# Autodesk Inventor assembly: 00090C
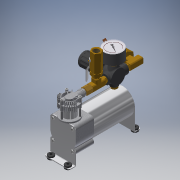
[picture p0: Inventor's stored thumbnail of the model, 180x180]
Saved by Autodesk Inventor 2016 (Build 200138000, 138)
## iProperties
Category: Pneumatics
Company: Autodesk Inc.
Created: 2015-12-06
Part Number: 00090C
Document SubType Name: Assembly
Designer: Autodesk Inc.
Catalog Web Link: http://www.viaircorp.com/OffRoad/90C.html
Description: Air Compressor 90C
Vendor: VIAIR
Author: Autodesk Inc.
## Documents named in this file (18)
- E:\Improved  2011 Robot\FRC KOP 2016\Pneumatics\Pneu_Compressor_0090C.iam
- E:\Improved  2011 Robot\FRC KOP 2016\Pneumatics\Parts\Pneumatics_VIAIR_0090_01.ipt
- E:\Improved  2011 Robot\FRC KOP 2016\Pneumatics\Parts\Pneumatics_VIAIR_0090_02.ipt
- E:\Improved  2011 Robot\FRC KOP 2016\Pneumatics\Parts\Pneumatics_VIAIR_00090_03.ipt
- E:\Improved  2011 Robot\FRC KOP 2016\Pneumatics\Parts\Pneumatics_VIAIR_0090_04.ipt
- E:\Improved  2011 Robot\FRC KOP 2016\Pneumatics\Parts\Union_62C-2.ipt
- E:\Improved  2011 Robot\FRC KOP 2016\Pneumatics\Parts\Pneumatic_VIAIR_Fitting.ipt
- E:\Improved  2011 Robot\FRC KOP 2016\Pneumatics\Parts\Pneumatics_VIAIR_00090_02.ipt
- E:\Improved  2011 Robot\FRC KOP 2016\Miscellaneous\Parts\ANSI B18.3 - 5-40 UNC - 1.5(31).ipt
- E:\Improved  2011 Robot\FRC KOP 2016\Miscellaneous\Parts\ANSI B18.3 - 6-32 UNC - UNC - 0.25(1).ipt
- E:\Improved  2011 Robot\FRC KOP 2016\Miscellaneous\Parts\ANSI B18.6.3 - 8-32 UNC - 1.25(30).ipt
- E:\Improved  2011 Robot\FRC KOP 2016\Pneumatics\Parts\Pneumatic_VIAIAR_00090_05.ipt
- E:\Improved  2011 Robot\FRC KOP 2016\Pneumatics\Pneu_Norgren_R07-100-RNEA.iam
- E:\Improved  2011 Robot\FRC KOP 2016\Pneumatics\Pneu_Plug_218P-2.ipt
- E:\Improved  2011 Robot\FRC KOP 2016\Pneumatics\Pneu_Parker_MV709-2.ipt
- E:\Improved  2011 Robot\FRC KOP 2016\Pneumatics\Pneu_Switch_SM-2B-115R.ipt
- E:\Improved  2011 Robot\FRC KOP 2016\Pneumatics\fc16-104_7.ipt
- E:\Improved  2011 Robot\FRC KOP 2016\Pneumatics\Pneu_Nipple_216P-2.ipt
## Components (29 placed, 17 different names)
1. Pneumatics_VIAIR_0090_01:1 — Mate:1, Flush:1, Flush:2, Mate:4, Angle:1, Mate:14, Mate:15, Mate:16, Mate:17, Mate:18, Mate:19, Mate:20, Mate:21, Angle:3, Mate:23, Mate:24, Flush:9, Flush:10, Mate:30, Mate:31
2. Pneumatics_VIAIR_0090_02:1 — Mate:1, Flush:1, Flush:2, Flush:3, Mate:2, Mate:3, Angle:2, Mate:29
3. Pneumatics_VIAIR_00090_03:1 — Flush:3, Mate:27, Mate:28, Mate:29
4. Pneumatics_VIAIR_0090_04:1 — Mate:2, Mate:3, Angle:2, Mate:6, Mate:7, Mate:8, Mate:9, Mate:10, Mate:11, Mate:12, Mate:13
5. Union_62C-2:1
6. Pneumatic_VIAIR_Fitting:1 — Mate:6, Mate:7, Mate:38, Mate:39
7. Pneumatics_VIAIR_00090_02:1 — Insert:1, Insert:2, Mate:25, Mate:26, Mate:27, Mate:28, Flush:9, Flush:10, Angle:4, Mate:32, Mate:33
8. Hexagon Socket Head Cap Screw - Inch No. 5 - 40 UNC - 1 1/2:1 — Mate:8, Mate:9
9. Hexagon Socket Head Cap Screw - Inch No. 5 - 40 UNC - 1 1/2:2 — Mate:10, Mate:11
10. Hexagon Socket Head Cap Screw - Inch No. 5 - 40 UNC - 1 1/2:3 — Mate:12, Mate:13
11. Hexagon Socket Button Head Cap Screw - Inch 6 - 32 x 1/4:1 — Mate:14, Mate:15
12. Hexagon Socket Button Head Cap Screw - Inch 6 - 32 x 1/4:2 — Mate:16, Mate:17
13. Hexagon Socket Button Head Cap Screw - Inch 6 - 32 x 1/4:3 — Mate:18, Mate:19
14. Hexagon Socket Button Head Cap Screw - Inch 6 - 32 x 1/4:4 — Mate:20, Mate:21
15. Indented Large Hex Head Machine Screw - Inch 8-32 UNC - 1.25:1 — Insert:1
16. Indented Large Hex Head Machine Screw - Inch 8-32 UNC - 1.25:2 — Insert:2
17. Pneumatic_VIAIAR_00090_05:1 — Mate:23, Mate:24
18. Pneumatic_VIAIAR_00090_05:2 — Mate:25, Mate:26, Angle:4
19. Pneumatic_VIAIAR_00090_05:3 — Mate:30, Mate:31
20. Pneumatic_VIAIAR_00090_05:4 — Mate:32, Mate:33
21. Pneu_Norgren_R07-100-RNEA:1 [sub-assembly] — Mate:36, Mate:37, Mate:43, Mate:44, Mate:49, Mate:50
22. Pneu_Plug_218P-2:1 — Mate:36, Mate:37
23. Pneu_Parker_MV709-2:1 — Mate:47, Mate:48
24. Pneu_Switch_SM-2B-115R:1 — Mate:53, Mate:54
25. fc16-104_7:1 — Mate:38, Mate:39, Mate:40, Mate:41, Mate:42, Mate:45, Mate:46
26. fc16-104_7:2 — Mate:51, Mate:52, Mate:53, Mate:54
27. Pneu_Nipple_216P-2:1 — Mate:40, Mate:41, Mate:42, Mate:43, Mate:44
28. Pneu_Nipple_216P-2:2 — Mate:45, Mate:46, Mate:47, Mate:48
29. Pneu_Nipple_216P-2:3 — Mate:49, Mate:50, Mate:51, Mate:52
## Relationships (64: Mate 52, Flush 6, Angle 4, Insert 2)
- Mate:1: Pneumatics_VIAIR_0090_01:1 ↔ Pneumatics_VIAIR_0090_02:1
- Flush:1: Pneumatics_VIAIR_0090_01:1 ↔ Pneumatics_VIAIR_0090_02:1
- Flush:2: Pneumatics_VIAIR_0090_01:1 ↔ Pneumatics_VIAIR_0090_02:1
- Flush:3: Pneumatics_VIAIR_0090_02:1 ↔ Pneumatics_VIAIR_00090_03:1
- Mate:2: Pneumatics_VIAIR_0090_02:1 ↔ Pneumatics_VIAIR_0090_04:1
- Mate:3: Pneumatics_VIAIR_0090_02:1 ↔ Pneumatics_VIAIR_0090_04:1
- Mate:4: Pneumatics_VIAIR_0090_01:1
- Mate:5
- Angle:1 (90 deg): Pneumatics_VIAIR_0090_01:1
- Flush:5 (-69.977 mm)
- Angle:2 (0 deg): Pneumatics_VIAIR_0090_02:1 ↔ Pneumatics_VIAIR_0090_04:1
- Mate:6: Pneumatics_VIAIR_0090_04:1 ↔ Pneumatic_VIAIR_Fitting:1
- Mate:7 (1.27 mm): Pneumatics_VIAIR_0090_04:1 ↔ Pneumatic_VIAIR_Fitting:1
- Mate:9: Pneumatics_VIAIR_0090_04:1 ↔ Hexagon Socket Head Cap Screw - Inch No. 5 - 40 UNC - 1 1/2:1
- Mate:11: Pneumatics_VIAIR_0090_04:1 ↔ Hexagon Socket Head Cap Screw - Inch No. 5 - 40 UNC - 1 1/2:2
- Mate:13: Pneumatics_VIAIR_0090_04:1 ↔ Hexagon Socket Head Cap Screw - Inch No. 5 - 40 UNC - 1 1/2:3
- Mate:15: Pneumatics_VIAIR_0090_01:1 ↔ Hexagon Socket Button Head Cap Screw - Inch 6 - 32 x 1/4:1
- Mate:17: Pneumatics_VIAIR_0090_01:1 ↔ Hexagon Socket Button Head Cap Screw - Inch 6 - 32 x 1/4:2
- Mate:19: Pneumatics_VIAIR_0090_01:1 ↔ Hexagon Socket Button Head Cap Screw - Inch 6 - 32 x 1/4:3
- Mate:21: Pneumatics_VIAIR_0090_01:1 ↔ Hexagon Socket Button Head Cap Screw - Inch 6 - 32 x 1/4:4
- Insert:1: Pneumatics_VIAIR_00090_02:1 ↔ Indented Large Hex Head Machine Screw - Inch 8-32 UNC - 1.25:1
- Insert:2: Pneumatics_VIAIR_00090_02:1 ↔ Indented Large Hex Head Machine Screw - Inch 8-32 UNC - 1.25:2
- Mate:22
- Angle:3 (90 deg): Pneumatics_VIAIR_0090_01:1
- Mate:23 (18.034 mm): Pneumatics_VIAIR_0090_01:1 ↔ Pneumatic_VIAIAR_00090_05:1
- Mate:24: Pneumatics_VIAIR_0090_01:1 ↔ Pneumatic_VIAIAR_00090_05:1
- Mate:25: Pneumatics_VIAIR_00090_02:1 ↔ Pneumatic_VIAIAR_00090_05:2
- Mate:26: Pneumatics_VIAIR_00090_02:1 ↔ Pneumatic_VIAIAR_00090_05:2
- Mate:27: Pneumatics_VIAIR_00090_03:1 ↔ Pneumatics_VIAIR_00090_02:1
- Mate:28: Pneumatics_VIAIR_00090_03:1 ↔ Pneumatics_VIAIR_00090_02:1
- Mate:29: Pneumatics_VIAIR_0090_02:1 ↔ Pneumatics_VIAIR_00090_03:1
- Flush:9: Pneumatics_VIAIR_0090_01:1 ↔ Pneumatics_VIAIR_00090_02:1
- Flush:10: Pneumatics_VIAIR_0090_01:1 ↔ Pneumatics_VIAIR_00090_02:1
- Angle:4 (0 deg): Pneumatics_VIAIR_00090_02:1 ↔ Pneumatic_VIAIAR_00090_05:2
- Mate:30: Pneumatics_VIAIR_0090_01:1 ↔ Pneumatic_VIAIAR_00090_05:3
- Mate:31: Pneumatics_VIAIR_0090_01:1 ↔ Pneumatic_VIAIAR_00090_05:3
- Mate:32: Pneumatics_VIAIR_00090_02:1 ↔ Pneumatic_VIAIAR_00090_05:4
- Mate:33: Pneumatics_VIAIR_00090_02:1 ↔ Pneumatic_VIAIAR_00090_05:4
- Mate:8: Pneumatics_VIAIR_0090_04:1 ↔ Hexagon Socket Head Cap Screw - Inch No. 5 - 40 UNC - 1 1/2:1
- Mate:10: Pneumatics_VIAIR_0090_04:1 ↔ Hexagon Socket Head Cap Screw - Inch No. 5 - 40 UNC - 1 1/2:2
- Mate:12: Pneumatics_VIAIR_0090_04:1 ↔ Hexagon Socket Head Cap Screw - Inch No. 5 - 40 UNC - 1 1/2:3
- Mate:14: Pneumatics_VIAIR_0090_01:1 ↔ Hexagon Socket Button Head Cap Screw - Inch 6 - 32 x 1/4:1
- Mate:16: Pneumatics_VIAIR_0090_01:1 ↔ Hexagon Socket Button Head Cap Screw - Inch 6 - 32 x 1/4:2
- Mate:18: Pneumatics_VIAIR_0090_01:1 ↔ Hexagon Socket Button Head Cap Screw - Inch 6 - 32 x 1/4:3
- Mate:20: Pneumatics_VIAIR_0090_01:1 ↔ Hexagon Socket Button Head Cap Screw - Inch 6 - 32 x 1/4:4
- Mate:36: Pneu_Norgren_R07-100-RNEA:1 ↔ Pneu_Plug_218P-2:1
- Mate:37: Pneu_Norgren_R07-100-RNEA:1 ↔ Pneu_Plug_218P-2:1
- Mate:38: Pneumatic_VIAIR_Fitting:1 ↔ fc16-104_7:1
- Mate:39: Pneumatic_VIAIR_Fitting:1 ↔ fc16-104_7:1
- Mate:40: fc16-104_7:1 ↔ Pneu_Nipple_216P-2:1
- Mate:41: fc16-104_7:1 ↔ Pneu_Nipple_216P-2:1
- Mate:42: fc16-104_7:1 ↔ Pneu_Nipple_216P-2:1
- Mate:43: Pneu_Norgren_R07-100-RNEA:1 ↔ Pneu_Nipple_216P-2:1
- Mate:44: Pneu_Norgren_R07-100-RNEA:1 ↔ Pneu_Nipple_216P-2:1
- Mate:45: fc16-104_7:1 ↔ Pneu_Nipple_216P-2:2
- Mate:46: fc16-104_7:1 ↔ Pneu_Nipple_216P-2:2
- Mate:47: Pneu_Parker_MV709-2:1 ↔ Pneu_Nipple_216P-2:2
- Mate:48: Pneu_Parker_MV709-2:1 ↔ Pneu_Nipple_216P-2:2
- Mate:49: Pneu_Norgren_R07-100-RNEA:1 ↔ Pneu_Nipple_216P-2:3
- Mate:50: Pneu_Norgren_R07-100-RNEA:1 ↔ Pneu_Nipple_216P-2:3
- Mate:51: fc16-104_7:2 ↔ Pneu_Nipple_216P-2:3
- Mate:52: fc16-104_7:2 ↔ Pneu_Nipple_216P-2:3
- Mate:53: Pneu_Switch_SM-2B-115R:1 ↔ fc16-104_7:2
- Mate:54: Pneu_Switch_SM-2B-115R:1 ↔ fc16-104_7:2
